# Autodesk Inventor assembly: pld_nipple
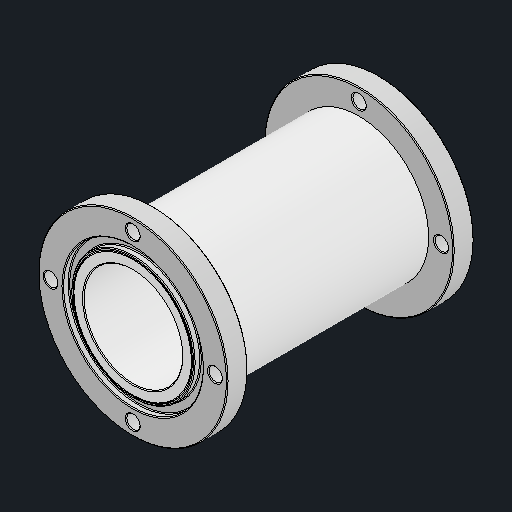
[picture p0: Inventor's stored thumbnail of the model, 512x512]
Saved by Autodesk Inventor 2026 (Build 300175050, 175E)
## iProperties
Created: 2025-11-12
Part Number: pld_nipple
Document SubType Name: Assembly
Designer: queezz
Author: queezz
## Documents named in this file (5)
- C:\Users\queezz\Dropbox\Drawings\PIHTI\PLD\pld_nipple.iam
- C:\Users\queezz\Dropbox\Drawings\PIHTI\PLD\pld_pipe.ipt
- C:\Users\queezz\Dropbox\Drawings\PIHTI\PLD\pld_flange_flat_ak.ipt
- C:\Users\queezz\Dropbox\Drawings\PIHTI\PLD\pld_flange_groove_ak.ipt
- C:\Users\queezz\Dropbox\Drawings\PIHTI\ContentCenter\Fastners\M6-nut.ipt
## Components (7 placed, 4 different names)
1. pld_pipe:1 — Rigid:1, Rigid:2, Mate:2
2. pld_flange_flat_ak:1 — Rigid:1, Mate:1, Rigid:3, Rigid:4, Rigid:5, Rigid:6
3. pld_flange_groove_ak:1 — Rigid:2
4. AS 1112 (4) - Metric M6:1 — Rigid:4
5. AS 1112 (4) - Metric M6:2 — Rigid:5
6. AS 1112 (4) - Metric M6:3 — Rigid:3
7. AS 1112 (4) - Metric M6:4 — Rigid:6
## Relationships (8: WeldJoint 6, Mate 2)
- Rigid:1 [WeldJoint]: pld_pipe:1 ↔ pld_flange_flat_ak:1
- Rigid:2 [WeldJoint]: pld_pipe:1 ↔ pld_flange_groove_ak:1
- Mate:1: pld_flange_flat_ak:1
- Mate:2: pld_pipe:1
- Rigid:3 [WeldJoint]: pld_flange_flat_ak:1 ↔ AS 1112 (4) - Metric M6:3
- Rigid:4 [WeldJoint]: pld_flange_flat_ak:1 ↔ AS 1112 (4) - Metric M6:1
- Rigid:5 [WeldJoint]: pld_flange_flat_ak:1 ↔ AS 1112 (4) - Metric M6:2
- Rigid:6 [WeldJoint]: pld_flange_flat_ak:1 ↔ AS 1112 (4) - Metric M6:4
